# Autodesk Inventor assembly: CCM_Unit_D
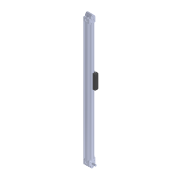
[picture p0: Inventor's stored thumbnail of the model, 180x180]
Saved by Autodesk Inventor 2020 (Build 240168000, 168)
## iProperties
Created: 2021-02-24
Part Number: CCM_Unit_D
Document SubType Name: Assembly
Designer: magnarecta
Author: magnarecta
## Documents named in this file (5)
- D:\Document\Github\Eto_Project\Hardware\Parts\CCM\CCM motion linear guide rail\CCM_UNIT\CCM_Unit_D.iam
- D:\Document\Github\Eto_Project\Hardware\Parts\CCM\CCM motion linear guide rail\CCM_UNIT\RAIL W40-06_B_MIR.ipt
- D:\Document\Github\Eto_Project\Hardware\Parts\CCM\CCM motion linear guide rail\CCM_UNIT\TAILSTOCK W40-00_0+0_MIR.ipt
- D:\Document\Github\Eto_Project\Hardware\Parts\CCM\CCM motion linear guide rail\CCM_UNIT\CART HK32-06W-00__1_MIR.ipt
- D:\Document\Github\Eto_Project\Hardware\Parts\CCM\CCM motion linear guide rail\CCM_UNIT\TAILSTOCK W40-00_0+22_1_MIR.ipt
## Components (4 placed, 4 different names)
1. RAIL W40-06_B_MIR:1 — フラッシュ:7, フラッシュ:8, メイト:4, フラッシュ:9, フラッシュ:10, メイト:5, スライダ:2
2. TAILSTOCK W40-00_0+0_MIR:1 — フラッシュ:7, フラッシュ:8, メイト:4
3. CART HK32-06W-00__1_MIR:1 — スライダ:2
4. TAILSTOCK W40-00_0+22_1_MIR:1 — フラッシュ:9, フラッシュ:10, メイト:5
## Relationships (7: Flush 4, Mate 2, TranslationJoint 1)
- フラッシュ:7 [Flush]: RAIL W40-06_B_MIR:1 ↔ TAILSTOCK W40-00_0+0_MIR:1
- フラッシュ:8 [Flush]: RAIL W40-06_B_MIR:1 ↔ TAILSTOCK W40-00_0+0_MIR:1
- メイト:4 [Mate]: RAIL W40-06_B_MIR:1 ↔ TAILSTOCK W40-00_0+0_MIR:1
- フラッシュ:9 [Flush]: RAIL W40-06_B_MIR:1 ↔ TAILSTOCK W40-00_0+22_1_MIR:1
- フラッシュ:10 [Flush]: RAIL W40-06_B_MIR:1 ↔ TAILSTOCK W40-00_0+22_1_MIR:1
- メイト:5 [Mate]: RAIL W40-06_B_MIR:1 ↔ TAILSTOCK W40-00_0+22_1_MIR:1
- スライダ:2 [TranslationJoint]: RAIL W40-06_B_MIR:1 ↔ CART HK32-06W-00__1_MIR:1
